# Autodesk Inventor assembly: Сборка1
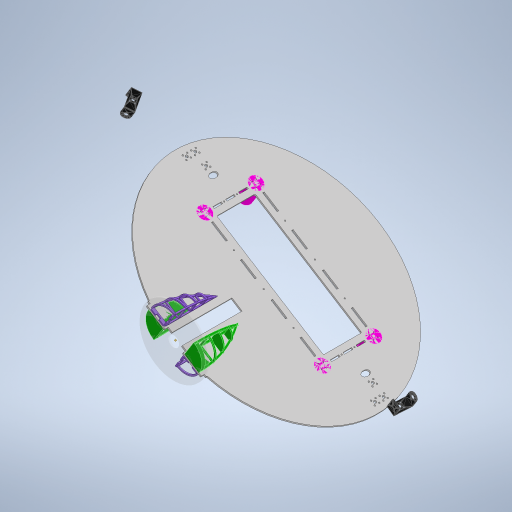
[picture p0: Inventor's stored thumbnail of the model, 512x512]
Saved by Autodesk Inventor 2023 (Build 270158000, 158)
## iProperties
Created: 2025-02-03
Part Number: Сборка1
Document SubType Name: Assembly
Designer: baranovaem
Author: baranovaem
## Documents named in this file (10)
- D:\лицо\Сборка1.iam
- D:\лицо\лицо1.ipt
- D:\лицо\магнит_стойка.ipt
- D:\лицо\монитор.ipt
- C:\Users\baranovaem\Downloads\экс\стенка.ipt
- D:\лицо\основа_лица.ipt
- D:\лицо\парус1.ipt
- D:\лицо\стенкаB.ipt
- \\sch239.net\UserHomes\Students\other\baranovaem\cheburashka\Cheburashka-main\Cheburashka_construction\korpus\acc1.ipt
- \\sch239.net\UserHomes\Students\other\baranovaem\cheburashka\Cheburashka-main\Cheburashka_construction\korpus\парус2.ipt
## Components (15 placed, 9 different names)
1. лицо1:1 — Совмещение:1, Совмещение:2, Угол:1, Совмещение:21, Совмещение:22, Совмещение:67, Совмещение:68, Совмещение:69, Совмещение:70
2. магнит_стойка:1
3. магнит_стойка:2 — Совмещение:32, Касательность:1
4. магнит_стойка:3 — Касательность:2
5. магнит_стойка:4
6. монитор:1 — Совмещение:32, Касательность:1, Касательность:2
7. стенка:1 — Совмещение:60, Совмещение:61
8. основа_лица:1 — Совмещение:21, Совмещение:22, Совмещение:58, Совмещение:59, Совмещение:60, Совмещение:61, Совмещение:62, Совмещение:63, Совмещение:64, Совмещение:65, Совмещение:66
9. парус1:2 — Совмещение:67, Совмещение:68
10. парус1:4 — Совмещение:69, Совмещение:70
11. стенкаB:1 — Совмещение:58, Совмещение:59
12. acc1:1 — Совмещение:62
13. acc1:2 — Совмещение:63
14. парус2:1 — Совмещение:64, Совмещение:65
15. парус2:2 — Совмещение:66
## Relationships (21: Mate 18, Tangent 2, Angle 1)
- Совмещение:1 [Mate]: лицо1:1
- Совмещение:2 [Mate]: лицо1:1
- Угол:1 [Angle] (0 deg): лицо1:1
- Совмещение:21 [Mate]: лицо1:1 ↔ основа_лица:1
- Совмещение:22 [Mate]: лицо1:1 ↔ основа_лица:1
- Совмещение:32 [Mate]: магнит_стойка:2 ↔ монитор:1
- Касательность:1 [Tangent]: магнит_стойка:2 ↔ монитор:1
- Касательность:2 [Tangent]: магнит_стойка:3 ↔ монитор:1
- Совмещение:58 [Mate]: основа_лица:1 ↔ стенкаB:1
- Совмещение:59 [Mate]: основа_лица:1 ↔ стенкаB:1
- Совмещение:60 [Mate]: стенка:1 ↔ основа_лица:1
- Совмещение:61 [Mate]: стенка:1 ↔ основа_лица:1
- Совмещение:62 [Mate]: основа_лица:1 ↔ acc1:1
- Совмещение:63 [Mate]: основа_лица:1 ↔ acc1:2
- Совмещение:64 [Mate]: основа_лица:1 ↔ парус2:1
- Совмещение:65 [Mate]: основа_лица:1 ↔ парус2:1
- Совмещение:66 [Mate]: основа_лица:1 ↔ парус2:2
- Совмещение:67 [Mate]: лицо1:1 ↔ парус1:2
- Совмещение:68 [Mate]: лицо1:1 ↔ парус1:2
- Совмещение:69 [Mate]: лицо1:1 ↔ парус1:4
- Совмещение:70 [Mate]: лицо1:1 ↔ парус1:4
